# Autodesk Inventor assembly: Ensamblaje1
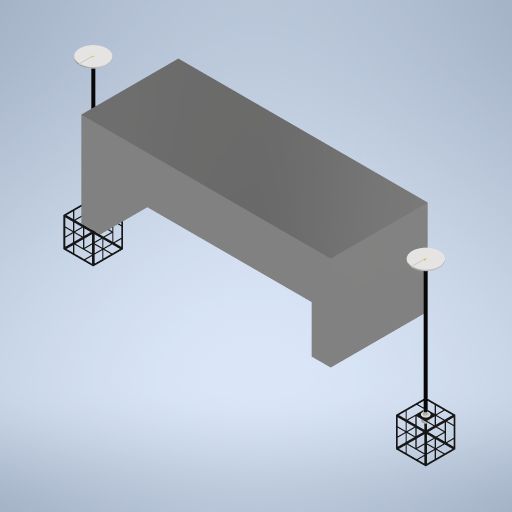
[picture p0: Inventor's stored thumbnail of the model, 512x512]
Saved by Autodesk Inventor 2024 (Build 280153000, 153)
## iProperties
Created: 2023-11-25
Part Number: Ensamblaje1
Document SubType Name: Assembly
Designer: sergi
Author: sergi
## Documents named in this file (8)
- C:\Users\sergi\OneDrive\Escritorio\proyectos\LamparaSalon\Ensamblaje1.iam
- C:\Users\sergi\OneDrive\Escritorio\proyectos\LamparaSalon\Barra.ipt
- C:\Users\sergi\OneDrive\Escritorio\proyectos\LamparaSalon\Processed_Acople E27.ipt
- C:\Users\sergi\OneDrive\Escritorio\proyectos\LamparaSalon\Casquillo.ipt
- C:\Users\sergi\OneDrive\Escritorio\proyectos\LamparaSalon\Pie.ipt
- C:\Users\sergi\OneDrive\Escritorio\proyectos\LamparaSalon\sofa.ipt
- C:\Users\sergi\OneDrive\Escritorio\proyectos\LamparaSalon\Pie2.ipt
- C:\Users\sergi\OneDrive\Escritorio\proyectos\LamparaSalon\EnsamblajeLampara.iam
## Components (11 placed, 7 different names)
1. Barra:1 — Coincidencia:1, Nivelación:1, Coincidencia:2, Nivelación:2, Coincidencia:4, Coincidencia:5, Nivelación:5
2. Processed_Acople E27:1 — Coincidencia:1, Nivelación:1, Coincidencia:3
3. Casquillo:1 — Coincidencia:2, Coincidencia:3
4. Pie:1 — Nivelación:2, Coincidencia:4, Nivelación:3, Nivelación:4
5. sofa:1 — Nivelación:3, Nivelación:8
6. Pie2:1 — Nivelación:4
7. EnsamblajeLampara:1 [sub-assembly] — Coincidencia:5, Nivelación:5
8. Barra:2 — Coincidencia:8, Coincidencia:9
9. Processed_Acople E27:2
10. Pie2:2 — Nivelación:8, Coincidencia:8, Coincidencia:9
11. EnsamblajeLampara:2 [sub-assembly]
## Relationships (17: Mate 9, Flush 8)
- Coincidencia:1 [Mate]: Barra:1 ↔ Processed_Acople E27:1
- Nivelación:1 [Flush]: Barra:1 ↔ Processed_Acople E27:1
- Coincidencia:2 [Mate]: Barra:1 ↔ Casquillo:1
- Coincidencia:3 [Mate]: Processed_Acople E27:1 ↔ Casquillo:1
- Nivelación:2 [Flush]: Barra:1 ↔ Pie:1
- Coincidencia:4 [Mate]: Barra:1 ↔ Pie:1
- Nivelación:3 [Flush]: Pie:1 ↔ sofa:1
- Nivelación:4 [Flush]: Pie:1 ↔ Pie2:1
- Coincidencia:5 [Mate]: Barra:1 ↔ EnsamblajeLampara:1
- Nivelación:5 [Flush]: Barra:1 ↔ EnsamblajeLampara:1
- [Mate]: Barra:2 ↔ Processed_Acople E27:2
- [Flush]: Barra:2 ↔ Processed_Acople E27:2
- [Mate]: Barra:2 ↔ EnsamblajeLampara:2
- [Flush]: Barra:2 ↔ EnsamblajeLampara:2
- Nivelación:8 [Flush]: sofa:1 ↔ Pie2:2
- Coincidencia:8 [Mate]: Barra:2 ↔ Pie2:2
- Coincidencia:9 [Mate]: Barra:2 ↔ Pie2:2
## Named parameters: d40_d4 = 0 mm, d41_d5 = 0 mm, d42_d38 = 0 mm, d43_d39 = 0 mm
